# Autodesk Inventor assembly: Z assembly
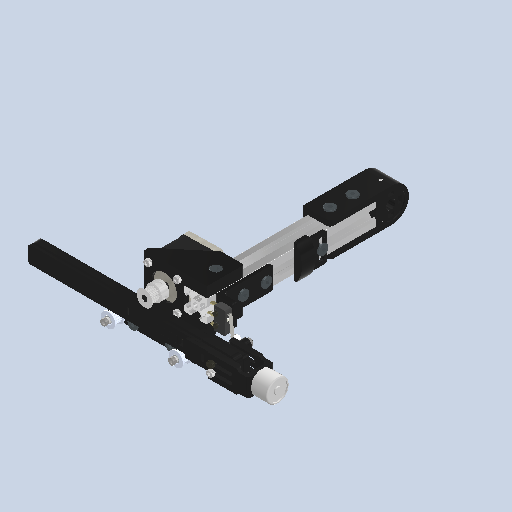
[picture p0: Inventor's stored thumbnail of the model, 512x512]
Saved by Autodesk Inventor 2022 (Build 260153000, 153)
## iProperties
Created: 2022-03-06
Part Number: Z assembly
Document SubType Name: Assembly
Designer: JK
Author: JK
## Documents named in this file (34)
- C:\Users\JK\Documents\Inventor\ScaraNema\SCARA-3DP\Parts\Forearm\Forearm assembly.iam
- C:\Users\JK\Documents\Inventor\ScaraNema\SCARA-3DP\Parts\Forearm\Z Motor support.ipt
- C:\Users\JK\Documents\Inventor\ScaraNema\SCARA-3DP\Parts\V-Slot 20x20.ipt
- C:\Users\JK\Documents\Inventor\ScaraNema\SCARA-3DP\Parts\Forearm\Z axis limit switch support.ipt
- C:\Users\JK\Documents\Inventor\ScaraNema\SCARA-3DP\Parts\Common components\V-Slot 20x20\V-Slot 20x20x150.ipt
- C:\Users\JK\Documents\Inventor\ScaraNema\SCARA-3DP\Parts\Forearm\Forearm support.ipt
- C:\Users\JK\Documents\Inventor\ScaraNema\SCARA-3DP\Parts\Common components\Limit switch.ipt
- C:\Users\JK\Documents\Inventor\ScaraNema\SCARA-3DP\Parts\Fasteners\M2x10 socket bolt.ipt
- C:\Users\JK\Documents\Inventor\ScaraNema\SCARA-3DP\Parts\Fasteners\M2 Hex nut.ipt
- C:\Users\JK\Documents\Inventor\ScaraNema\SCARA-3DP\Parts\Fasteners\M3x10 set screw.ipt
- C:\Users\JK\Documents\Inventor\ScaraNema\SCARA-3DP\Parts\Fasteners\M5x15 Flat head bolt.ipt
- C:\Users\JK\Documents\Inventor\ScaraNema\SCARA-3DP\Parts\Fasteners\M5x10 Flat head bolt.ipt
- C:\Users\JK\Documents\Inventor\ScaraNema\SCARA-3DP\Parts\Fasteners\M5x8 Flat head bolt.ipt
- C:\Users\JK\Documents\Inventor\ScaraNema\SCARA-3DP\Parts\Fasteners\M3 Hex nut.ipt
- C:\Users\JK\Documents\Inventor\ScaraNema\SCARA-3DP\Parts\Fasteners\M5 T-Nut Drop-in 20x20.ipt
- C:\Users\JK\Documents\Inventor\ScaraNema\SCARA-3DP\Parts\Fasteners\M3x6 socket bolt.ipt
- C:\Users\JK\Documents\Inventor\ScaraNema\SCARA-3DP\Parts\Forearm\Arm endstop.ipt
- C:\Users\JK\Documents\Inventor\ScaraNema\SCARA-3DP\Parts\Forearm\Nema14 Stepper Motor v1.ipt
- C:\Users\JK\Documents\Inventor\ScaraNema\SCARA-3DP\Parts\Common components\GT2 16 Pulley.ipt
- C:\Users\JK\Documents\Inventor\ScaraNema\SCARA-3DP\Parts\Forearm\GT2RackA.ipt
- C:\Users\JK\Documents\Inventor\ScaraNema\SCARA-3DP\Parts\Forearm\Wedge.ipt
- C:\Users\JK\Documents\Inventor\ScaraNema\SCARA-3DP\Parts\Forearm\GT2RackB.ipt
- C:\Users\JK\Documents\Inventor\ScaraNema\SCARA-3DP\Parts\Forearm\Rack support.ipt
- C:\Users\JK\Documents\Inventor\ScaraNema\SCARA-3DP\Parts\Forearm\magnetsupport.ipt
- C:\Users\JK\Documents\Inventor\ScaraNema\SCARA-3DP\Parts\Common components\Idle pulley 16\GT2-16 Idle pulley.iam
- C:\Users\JK\Documents\Inventor\ScaraNema\SCARA-3DP\Parts\Fasteners\M3x35 socket bolt.ipt
- C:\Users\JK\Documents\Inventor\ScaraNema\SCARA-3DP\Parts\Forearm\m3separator.ipt
- C:\Users\JK\Documents\Inventor\ScaraNema\SCARA-3DP\Parts\Forearm\electromagnet.ipt
- C:\Users\JK\Documents\Inventor\ScaraNema\SCARA-3DP\Parts\Fasteners\M5 Hex nut.ipt
- C:\Users\JK\Documents\Inventor\ScaraNema\SCARA-3DP\Parts\Fasteners\M4x10 socket bolt.ipt
- C:\Users\JK\Documents\Inventor\ScaraNema\SCARA-3DP\Parts\Fasteners\M3x25 socket solt.ipt
- C:\Users\JK\Documents\Inventor\ScaraNema\SCARA-3DP\Parts\Forearm\small separator.ipt
- C:\Users\JK\Documents\Inventor\ScaraNema\SCARA-3DP\Parts\Fasteners\M3x20SocketBolt.ipt
- C:\Users\JK\Documents\Inventor\ScaraNema\SCARA-3DP\Parts\Fasteners\M3x30 socket bolt.ipt
## Components (71 placed, 32 different names)
1. Z Motor support:1 — Nivelación:1, Coincidencia:32, Coincidencia:48, Ángulo:19, Coincidencia:91, Coincidencia:92, Coincidencia:93, Coincidencia:94, Coincidencia:95, Coincidencia:96, Coincidencia:103, Coincidencia:104, Coincidencia:117, Tangente:2, Coincidencia:118, Coincidencia:129, Nivelación:29, Nivelación:31, Coincidencia:150, Coincidencia:151, Coincidencia:152, Ángulo:25, Ángulo:26
2. V-Slot 20x20x150:1 — Nivelación:1, Coincidencia:17, Coincidencia:18, Ángulo:12, Coincidencia:98, Coincidencia:100, Coincidencia:117, Coincidencia:132, Nivelación:30, Nivelación:31, Nivelación:32
3. Z axis limit switch support:1 — Ángulo:5, Coincidencia:28, Coincidencia:46, Coincidencia:47, Coincidencia:132, Nivelación:29, Nivelación:30, Coincidencia:133, Coincidencia:134, Ángulo:24, Coincidencia:136, Coincidencia:137, Nivelación:33, Coincidencia:149
4. Forearm support:1 — Coincidencia:17, Coincidencia:18, Coincidencia:33, Coincidencia:34, Coincidencia:35, Coincidencia:36, Coincidencia:37, Coincidencia:38, Coincidencia:42, Ángulo:8, Coincidencia:43, Coincidencia:44, Coincidencia:45, Ángulo:15, Coincidencia:83, Coincidencia:84, Coincidencia:85, Coincidencia:86, Coincidencia:88, Coincidencia:98, Coincidencia:99, Coincidencia:101, Ángulo:21
5. M2x10 socket bolt:1 — Nivelación:9, Coincidencia:26, Coincidencia:134
6. M2x10 socket bolt:2 — Nivelación:9, Coincidencia:27, Coincidencia:133, Coincidencia:138
7. M2 Hex nut:1 — Coincidencia:27, Nivelación:10, Ángulo:4, Ángulo:5
8. M2 Hex nut:2 — Coincidencia:26, Nivelación:10, Ángulo:4, Coincidencia:28
9. M5x15 Flat head bolt:1 — Coincidencia:32, Coincidencia:73, Coincidencia:93
10. M5x10 Flat head bolt:1 — Coincidencia:33, Nivelación:12, Coincidencia:82, Coincidencia:86
11. M5x10 Flat head bolt:2 — Coincidencia:34, Nivelación:12, Coincidencia:81
12. M5x10 Flat head bolt:3 — Coincidencia:35, Nivelación:11, Coincidencia:77, Coincidencia:88
13. M5x10 Flat head bolt:4 — Coincidencia:36, Nivelación:11, Coincidencia:78
14. M5x8 Flat head bolt:1 — Coincidencia:37, Nivelación:13, Coincidencia:79, Coincidencia:99
15. M5x8 Flat head bolt:2 — Coincidencia:38, Nivelación:13, Coincidencia:80
16. M5x8 Flat head bolt:3 — Coincidencia:47, Nivelación:15, Coincidencia:75, Coincidencia:149
17. M5x8 Flat head bolt:4 — Coincidencia:46, Nivelación:15, Coincidencia:74
18. M5x15 Flat head bolt:2 — Coincidencia:48, Coincidencia:76, Coincidencia:94
19. M5 T-Nut Drop-in 20x20:1 — Coincidencia:73, Coincidencia:91
20. M5 T-Nut Drop-in 20x20:2 — Coincidencia:74, Nivelación:22, Ángulo:18, Ángulo:19
21. M5 T-Nut Drop-in 20x20:3 — Coincidencia:75, Nivelación:22, Ángulo:18, Nivelación:33
22. M5 T-Nut Drop-in 20x20:4 — Coincidencia:76, Coincidencia:92
23. M5 T-Nut Drop-in 20x20:5 — Coincidencia:77, Ángulo:13, Nivelación:25, Ángulo:14, Ángulo:17, Coincidencia:84
24. M5 T-Nut Drop-in 20x20:6 — Coincidencia:78, Ángulo:13, Nivelación:25, Ángulo:14, Ángulo:15
25. M5 T-Nut Drop-in 20x20:7 — Coincidencia:79, Nivelación:23, Ángulo:11, Coincidencia:85
26. M5 T-Nut Drop-in 20x20:8 — Coincidencia:80, Nivelación:23, Ángulo:11, Ángulo:12
27. M5 T-Nut Drop-in 20x20:9 — Coincidencia:82, Nivelación:24, Ángulo:16, Coincidencia:83
28. M5 T-Nut Drop-in 20x20:10 — Coincidencia:81, Nivelación:24, Ángulo:16, Ángulo:17
29. Arm endstop:1 — Coincidencia:100, Coincidencia:101, Coincidencia:147, Coincidencia:148
30. Nema14 Stepper Motor v1:1 — Coincidencia:103, Coincidencia:104, Coincidencia:105, Nivelación:26
31. GT2 16 Pulley:1 — Coincidencia:105, Nivelación:26, Tangente:1, Coincidencia:116
32. GT2RackA:1 — Coincidencia:106, Ángulo:20, Coincidencia:107, Nivelación:27, Coincidencia:108, Coincidencia:109, Tangente:1, Coincidencia:116, Ángulo:22, Coincidencia:176, Coincidencia:177
33. Wedge:1 — Nivelación:27, Coincidencia:108, Coincidencia:109
34. GT2RackB:1 — Coincidencia:106, Ángulo:20, Coincidencia:107, Coincidencia:126, Ángulo:23, Coincidencia:130, Coincidencia:139, Coincidencia:159, Coincidencia:160, Ángulo:29, Ángulo:30, Coincidencia:161, Ángulo:31, Coincidencia:162, Coincidencia:163, Coincidencia:166
35. Rack support:1 — Tangente:2, Coincidencia:118, Ángulo:21, Ángulo:22, Coincidencia:127, Coincidencia:128, Coincidencia:129, Coincidencia:131, Coincidencia:155, Coincidencia:156, Coincidencia:157, Ángulo:27, Ángulo:28, Coincidencia:158
36. magnetsupport:1 — Coincidencia:126, Ángulo:23, Coincidencia:130, Coincidencia:140, Coincidencia:142, Coincidencia:143, Coincidencia:144, Coincidencia:164, Coincidencia:165, Coincidencia:167
37. GT2-16 Idle pulley:1 [sub-assembly] — Coincidencia:127, Nivelación:28, Coincidencia:131, Coincidencia:170
38. GT2-16 Idle pulley:2 [sub-assembly] — Coincidencia:128, Nivelación:28, Coincidencia:171, Coincidencia:172
39. Limit switch:2 — Ángulo:24, Coincidencia:136, Coincidencia:137, Coincidencia:138
40. M3x35 socket bolt:1 — Coincidencia:139, Coincidencia:140, Coincidencia:141, Coincidencia:168
41. m3separator:1 — Coincidencia:141, Coincidencia:142, Coincidencia:169
42. electromagnet:1 — Coincidencia:143, Coincidencia:144
43. M5x8 Flat head bolt:5 — Coincidencia:146, Coincidencia:147
44. M5 T-Nut Drop-in 20x20:11 — Coincidencia:146, Coincidencia:148, Nivelación:32
45. M5 Hex nut:1 — Coincidencia:150, Nivelación:34, Coincidencia:152, Ángulo:25, Coincidencia:153
46. M5 Hex nut:2 — Coincidencia:151, Nivelación:34, Ángulo:26, Coincidencia:154
47. M5x15 Flat head bolt:3 — Coincidencia:154, Nivelación:35
48. M5x15 Flat head bolt:4 — Coincidencia:153, Nivelación:35, Coincidencia:155
49. M3 Hex nut:6 — Coincidencia:157, Ángulo:27, Nivelación:36
50. M3 Hex nut:7 — Coincidencia:156, Ángulo:28, Coincidencia:158, Nivelación:36
51. M3 Hex nut:8 — Coincidencia:160, Ángulo:30, Nivelación:37
52. M3 Hex nut:9 — Coincidencia:159, Ángulo:29, Nivelación:37, Coincidencia:161
53. M3 Hex nut:10 — Ángulo:31, Coincidencia:162, Coincidencia:163
54. M4x10 socket bolt:1 — Coincidencia:164, Coincidencia:165
55. M3x25 socket solt:1 — Coincidencia:166, Coincidencia:167
56. M3 Hex nut:11 — Coincidencia:168, Coincidencia:169
57. small separator:1 — Coincidencia:170, Nivelación:38, Coincidencia:173, Coincidencia:175
58. small separator:2 — Coincidencia:171, Nivelación:38, Coincidencia:172, Coincidencia:174
59. M3x20SocketBolt:1 — Coincidencia:173, Nivelación:39, Coincidencia:175
60. M3x20SocketBolt:2 — Coincidencia:174, Nivelación:39
61. M3x30 socket bolt:1 — Coincidencia:176, Coincidencia:177
62. M3x10 set screw:5 — Coincidencia:44, Coincidencia:45
63. M3 Hex nut:1 — Coincidencia:42, Ángulo:8, Coincidencia:43
64. M3x10 set screw:6
65. M3 Hex nut:4
66. M3x10 set screw:7
67. M3 Hex nut:5
68. M3x6 socket bolt:2 — Coincidencia:95, Coincidencia:96
69. M3x6 socket bolt:3
70. M3x6 socket bolt:4
71. M3x6 socket bolt:5
## Component patterns: (3 elements, first: M3x10 set screw:5 + M3 Hex nut:1), (4 elements, first: M3x6 socket bolt:2)
## Relationships (155: Mate 104, Flush 25, Angle 24, Tangent 2)
- Nivelación:1 [Flush]: Z Motor support:1 ↔ V-Slot 20x20x150:1
- Coincidencia:17 [Mate]: V-Slot 20x20x150:1 ↔ Forearm support:1
- Coincidencia:18 [Mate] (0.15 mm): V-Slot 20x20x150:1 ↔ Forearm support:1
- Nivelación:9 [Flush]: M2x10 socket bolt:1 ↔ M2x10 socket bolt:2
- Coincidencia:26 [Mate]: M2x10 socket bolt:1 ↔ M2 Hex nut:2
- Coincidencia:27 [Mate]: M2x10 socket bolt:2 ↔ M2 Hex nut:1
- Nivelación:10 [Flush]: M2 Hex nut:1 ↔ M2 Hex nut:2
- Ángulo:4 [Angle] (0 deg): M2 Hex nut:1 ↔ M2 Hex nut:2
- Ángulo:5 [Angle] (0 deg): Z axis limit switch support:1 ↔ M2 Hex nut:1
- Coincidencia:28 [Mate]: Z axis limit switch support:1 ↔ M2 Hex nut:2
- Coincidencia:32 [Mate]: Z Motor support:1 ↔ M5x15 Flat head bolt:1
- Coincidencia:33 [Mate]: Forearm support:1 ↔ M5x10 Flat head bolt:1
- Coincidencia:34 [Mate]: Forearm support:1 ↔ M5x10 Flat head bolt:2
- Coincidencia:35 [Mate]: Forearm support:1 ↔ M5x10 Flat head bolt:3
- Coincidencia:36 [Mate]: Forearm support:1 ↔ M5x10 Flat head bolt:4
- Nivelación:11 [Flush]: M5x10 Flat head bolt:3 ↔ M5x10 Flat head bolt:4
- Nivelación:12 [Flush]: M5x10 Flat head bolt:1 ↔ M5x10 Flat head bolt:2
- Coincidencia:37 [Mate]: Forearm support:1 ↔ M5x8 Flat head bolt:1
- Coincidencia:38 [Mate]: Forearm support:1 ↔ M5x8 Flat head bolt:2
- Nivelación:13 [Flush]: M5x8 Flat head bolt:1 ↔ M5x8 Flat head bolt:2
- Coincidencia:42 [Mate]: Forearm support:1 ↔ M3 Hex nut:1
- Ángulo:8 [Angle] (0 deg): Forearm support:1 ↔ M3 Hex nut:1
- Coincidencia:43 [Mate]: Forearm support:1 ↔ M3 Hex nut:1
- Coincidencia:44 [Mate]: Forearm support:1 ↔ M3x10 set screw:5
- Coincidencia:45 [Mate] (-5 mm): Forearm support:1 ↔ M3x10 set screw:5
- Coincidencia:46 [Mate]: Z axis limit switch support:1 ↔ M5x8 Flat head bolt:4
- Coincidencia:47 [Mate]: Z axis limit switch support:1 ↔ M5x8 Flat head bolt:3
- Nivelación:15 [Flush]: M5x8 Flat head bolt:3 ↔ M5x8 Flat head bolt:4
- Coincidencia:48 [Mate]: Z Motor support:1 ↔ M5x15 Flat head bolt:2
- Coincidencia:73 [Mate]: M5x15 Flat head bolt:1 ↔ M5 T-Nut Drop-in 20x20:1
- Coincidencia:74 [Mate]: M5x8 Flat head bolt:4 ↔ M5 T-Nut Drop-in 20x20:2
- Coincidencia:75 [Mate]: M5x8 Flat head bolt:3 ↔ M5 T-Nut Drop-in 20x20:3
- Coincidencia:76 [Mate]: M5x15 Flat head bolt:2 ↔ M5 T-Nut Drop-in 20x20:4
- Nivelación:22 [Flush]: M5 T-Nut Drop-in 20x20:2 ↔ M5 T-Nut Drop-in 20x20:3
- Coincidencia:77 [Mate]: M5x10 Flat head bolt:3 ↔ M5 T-Nut Drop-in 20x20:5
- Coincidencia:78 [Mate]: M5x10 Flat head bolt:4 ↔ M5 T-Nut Drop-in 20x20:6
- Coincidencia:79 [Mate]: M5x8 Flat head bolt:1 ↔ M5 T-Nut Drop-in 20x20:7
- Coincidencia:80 [Mate]: M5x8 Flat head bolt:2 ↔ M5 T-Nut Drop-in 20x20:8
- Coincidencia:81 [Mate]: M5x10 Flat head bolt:2 ↔ M5 T-Nut Drop-in 20x20:10
- Coincidencia:82 [Mate]: M5x10 Flat head bolt:1 ↔ M5 T-Nut Drop-in 20x20:9
- Nivelación:23 [Flush]: M5 T-Nut Drop-in 20x20:7 ↔ M5 T-Nut Drop-in 20x20:8
- Nivelación:24 [Flush]: M5 T-Nut Drop-in 20x20:9 ↔ M5 T-Nut Drop-in 20x20:10
- Ángulo:11 [Angle] (0 deg): M5 T-Nut Drop-in 20x20:7 ↔ M5 T-Nut Drop-in 20x20:8
- Ángulo:12 [Angle] (90 deg): V-Slot 20x20x150:1 ↔ M5 T-Nut Drop-in 20x20:8
- Ángulo:13 [Angle] (0 deg): M5 T-Nut Drop-in 20x20:5 ↔ M5 T-Nut Drop-in 20x20:6
- Nivelación:25 [Flush]: M5 T-Nut Drop-in 20x20:5 ↔ M5 T-Nut Drop-in 20x20:6
- Ángulo:14 [Angle] (0 deg): M5 T-Nut Drop-in 20x20:5 ↔ M5 T-Nut Drop-in 20x20:6
- Ángulo:15 [Angle] (0 deg): Forearm support:1 ↔ M5 T-Nut Drop-in 20x20:6
- Ángulo:16 [Angle] (0 deg): M5 T-Nut Drop-in 20x20:9 ↔ M5 T-Nut Drop-in 20x20:10
- Ángulo:17 [Angle] (0 deg): M5 T-Nut Drop-in 20x20:5 ↔ M5 T-Nut Drop-in 20x20:10
- Coincidencia:83 [Mate] (0.6 mm): Forearm support:1 ↔ M5 T-Nut Drop-in 20x20:9
- Coincidencia:84 [Mate] (0.6 mm): Forearm support:1 ↔ M5 T-Nut Drop-in 20x20:5
- Coincidencia:85 [Mate] (0.6 mm): Forearm support:1 ↔ M5 T-Nut Drop-in 20x20:7
- Coincidencia:86 [Mate]: Forearm support:1 ↔ M5x10 Flat head bolt:1
- Coincidencia:88 [Mate]: Forearm support:1 ↔ M5x10 Flat head bolt:3
- Ángulo:18 [Angle] (0 deg): M5 T-Nut Drop-in 20x20:2 ↔ M5 T-Nut Drop-in 20x20:3
- Ángulo:19 [Angle] (0 deg): Z Motor support:1 ↔ M5 T-Nut Drop-in 20x20:2
- Coincidencia:91 [Mate] (0.6 mm): Z Motor support:1 ↔ M5 T-Nut Drop-in 20x20:1
- Coincidencia:92 [Mate] (0.6 mm): Z Motor support:1 ↔ M5 T-Nut Drop-in 20x20:4
- Coincidencia:93 [Mate]: Z Motor support:1 ↔ M5x15 Flat head bolt:1
- Coincidencia:94 [Mate]: Z Motor support:1 ↔ M5x15 Flat head bolt:2
- Coincidencia:95 [Mate]: Z Motor support:1 ↔ M3x6 socket bolt:2
- Coincidencia:96 [Mate]: Z Motor support:1 ↔ M3x6 socket bolt:2
- Coincidencia:98 [Mate]: V-Slot 20x20x150:1 ↔ Forearm support:1
- Coincidencia:99 [Mate]: Forearm support:1 ↔ M5x8 Flat head bolt:1
- Coincidencia:100 [Mate]: V-Slot 20x20x150:1 ↔ Arm endstop:1
- Coincidencia:101 [Mate] (20 mm): Forearm support:1 ↔ Arm endstop:1
- Coincidencia:103 [Mate]: Z Motor support:1 ↔ Nema14 Stepper Motor v1:1
- Coincidencia:104 [Mate]: Z Motor support:1 ↔ Nema14 Stepper Motor v1:1
- Coincidencia:105 [Mate]: Nema14 Stepper Motor v1:1 ↔ GT2 16 Pulley:1
- Nivelación:26 [Flush]: Nema14 Stepper Motor v1:1 ↔ GT2 16 Pulley:1
- Coincidencia:106 [Mate]: GT2RackA:1 ↔ GT2RackB:1
- Ángulo:20 [Angle] (0 deg): GT2RackA:1 ↔ GT2RackB:1
- Coincidencia:107 [Mate] (1 mm): GT2RackA:1 ↔ GT2RackB:1
- Nivelación:27 [Flush]: GT2RackA:1 ↔ Wedge:1
- Coincidencia:108 [Mate]: GT2RackA:1 ↔ Wedge:1
- Coincidencia:109 [Mate] (0.15 mm): GT2RackA:1 ↔ Wedge:1
- Tangente:1 (-0.5 mm): GT2 16 Pulley:1 ↔ GT2RackA:1
- Coincidencia:116 [Mate] (0.5 mm): GT2 16 Pulley:1 ↔ GT2RackA:1
- Coincidencia:117 [Mate] (0.15 mm): Z Motor support:1 ↔ V-Slot 20x20x150:1
- Tangente:2: Z Motor support:1 ↔ Rack support:1
- Coincidencia:118 [Mate]: Z Motor support:1 ↔ Rack support:1
- Ángulo:21 [Angle] (0 deg): Forearm support:1 ↔ Rack support:1
- Ángulo:22 [Angle] (0 deg): GT2RackA:1 ↔ Rack support:1
- Coincidencia:126 [Mate] (0.15 mm): GT2RackB:1 ↔ magnetsupport:1
- Ángulo:23 [Angle] (0 deg): GT2RackB:1 ↔ magnetsupport:1
- Coincidencia:127 [Mate]: Rack support:1 ↔ GT2-16 Idle pulley:1
- Coincidencia:128 [Mate]: Rack support:1 ↔ GT2-16 Idle pulley:2
- Nivelación:28 [Flush]: GT2-16 Idle pulley:1 ↔ GT2-16 Idle pulley:2
- Coincidencia:129 [Mate]: Z Motor support:1 ↔ Rack support:1
- Coincidencia:130 [Mate]: GT2RackB:1 ↔ magnetsupport:1
- Coincidencia:131 [Mate] (1.2 mm): Rack support:1 ↔ GT2-16 Idle pulley:1
- Coincidencia:132 [Mate]: V-Slot 20x20x150:1 ↔ Z axis limit switch support:1
- Nivelación:29 [Flush] (7 mm): Z Motor support:1 ↔ Z axis limit switch support:1
- Nivelación:30 [Flush]: V-Slot 20x20x150:1 ↔ Z axis limit switch support:1
- Nivelación:31 [Flush]: Z Motor support:1 ↔ V-Slot 20x20x150:1
- Coincidencia:133 [Mate]: Z axis limit switch support:1 ↔ M2x10 socket bolt:2
- Coincidencia:134 [Mate]: Z axis limit switch support:1 ↔ M2x10 socket bolt:1
- Ángulo:24 [Angle] (0 deg): Z axis limit switch support:1 ↔ Limit switch:2
- Coincidencia:136 [Mate]: Z axis limit switch support:1 ↔ Limit switch:2
- Coincidencia:137 [Mate]: Z axis limit switch support:1 ↔ Limit switch:2
- Coincidencia:138 [Mate]: M2x10 socket bolt:2 ↔ Limit switch:2
- Coincidencia:139 [Mate]: GT2RackB:1 ↔ M3x35 socket bolt:1
- Coincidencia:140 [Mate]: magnetsupport:1 ↔ M3x35 socket bolt:1
- Coincidencia:141 [Mate]: M3x35 socket bolt:1 ↔ m3separator:1
- Coincidencia:142 [Mate]: magnetsupport:1 ↔ m3separator:1
- Coincidencia:143 [Mate]: magnetsupport:1 ↔ electromagnet:1
- Coincidencia:144 [Mate]: magnetsupport:1 ↔ electromagnet:1
- Coincidencia:146 [Mate]: M5x8 Flat head bolt:5 ↔ M5 T-Nut Drop-in 20x20:11
- Coincidencia:147 [Mate]: Arm endstop:1 ↔ M5x8 Flat head bolt:5
- Coincidencia:148 [Mate] (1 mm): Arm endstop:1 ↔ M5 T-Nut Drop-in 20x20:11
- Nivelación:32 [Flush] (7 mm): V-Slot 20x20x150:1 ↔ M5 T-Nut Drop-in 20x20:11
- Nivelación:33 [Flush] (3 mm): Z axis limit switch support:1 ↔ M5 T-Nut Drop-in 20x20:3
- Coincidencia:149 [Mate]: Z axis limit switch support:1 ↔ M5x8 Flat head bolt:3
- Coincidencia:150 [Mate]: Z Motor support:1 ↔ M5 Hex nut:1
- Coincidencia:151 [Mate]: Z Motor support:1 ↔ M5 Hex nut:2
- Nivelación:34 [Flush]: M5 Hex nut:1 ↔ M5 Hex nut:2
- Coincidencia:152 [Mate]: Z Motor support:1 ↔ M5 Hex nut:1
- Ángulo:25 [Angle] (0 deg): Z Motor support:1 ↔ M5 Hex nut:1
- Ángulo:26 [Angle] (0 deg): Z Motor support:1 ↔ M5 Hex nut:2
- Coincidencia:153 [Mate]: M5 Hex nut:1 ↔ M5x15 Flat head bolt:4
- Coincidencia:154 [Mate]: M5 Hex nut:2 ↔ M5x15 Flat head bolt:3
- Nivelación:35 [Flush]: M5x15 Flat head bolt:3 ↔ M5x15 Flat head bolt:4
- Coincidencia:155 [Mate]: Rack support:1 ↔ M5x15 Flat head bolt:4
- Coincidencia:156 [Mate]: Rack support:1 ↔ M3 Hex nut:7
- Coincidencia:157 [Mate]: Rack support:1 ↔ M3 Hex nut:6
- Ángulo:27 [Angle] (0 deg): Rack support:1 ↔ M3 Hex nut:6
- Ángulo:28 [Angle] (0 deg): Rack support:1 ↔ M3 Hex nut:7
- Coincidencia:158 [Mate]: Rack support:1 ↔ M3 Hex nut:7
- Nivelación:36 [Flush]: M3 Hex nut:6 ↔ M3 Hex nut:7
- Coincidencia:159 [Mate]: GT2RackB:1 ↔ M3 Hex nut:9
- Coincidencia:160 [Mate]: GT2RackB:1 ↔ M3 Hex nut:8
- Ángulo:29 [Angle] (0 deg): GT2RackB:1 ↔ M3 Hex nut:9
- Ángulo:30 [Angle] (0 deg): GT2RackB:1 ↔ M3 Hex nut:8
- Nivelación:37 [Flush]: M3 Hex nut:8 ↔ M3 Hex nut:9
- Coincidencia:161 [Mate]: GT2RackB:1 ↔ M3 Hex nut:9
- Ángulo:31 [Angle] (0 deg): GT2RackB:1 ↔ M3 Hex nut:10
- Coincidencia:162 [Mate]: GT2RackB:1 ↔ M3 Hex nut:10
- Coincidencia:163 [Mate]: GT2RackB:1 ↔ M3 Hex nut:10
- Coincidencia:164 [Mate]: magnetsupport:1 ↔ M4x10 socket bolt:1
- Coincidencia:165 [Mate]: magnetsupport:1 ↔ M4x10 socket bolt:1
- Coincidencia:166 [Mate]: GT2RackB:1 ↔ M3x25 socket solt:1
- Coincidencia:167 [Mate]: magnetsupport:1 ↔ M3x25 socket solt:1
- Coincidencia:168 [Mate]: M3x35 socket bolt:1 ↔ M3 Hex nut:11
- Coincidencia:169 [Mate]: m3separator:1 ↔ M3 Hex nut:11
- Coincidencia:170 [Mate]: GT2-16 Idle pulley:1 ↔ small separator:1
- Coincidencia:171 [Mate]: GT2-16 Idle pulley:2 ↔ small separator:2
- Nivelación:38 [Flush]: small separator:1 ↔ small separator:2
- Coincidencia:172 [Mate]: GT2-16 Idle pulley:2 ↔ small separator:2
- Coincidencia:173 [Mate]: small separator:1 ↔ M3x20SocketBolt:1
- Coincidencia:174 [Mate]: small separator:2 ↔ M3x20SocketBolt:2
- Nivelación:39 [Flush]: M3x20SocketBolt:1 ↔ M3x20SocketBolt:2
- Coincidencia:175 [Mate]: small separator:1 ↔ M3x20SocketBolt:1
- Coincidencia:176 [Mate]: GT2RackA:1 ↔ M3x30 socket bolt:1
- Coincidencia:177 [Mate]: GT2RackA:1 ↔ M3x30 socket bolt:1
